# Autodesk Inventor assembly: SC40 700 Assembly
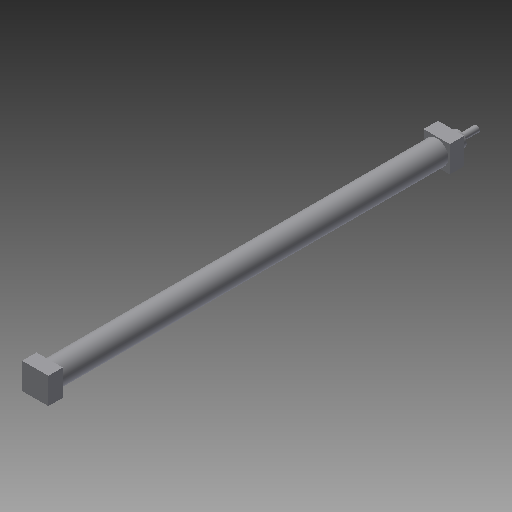
[picture p0: Inventor's stored thumbnail of the model, 512x512]
Saved by Autodesk Inventor 2019.4 (Build 234330000, 330)
## iProperties
Created: 2020-01-10
Part Number: SC40 700 Assembly
Document SubType Name: Assembly
Designer: Mark
Mass: 1404.85 g
Surface Area: 1514.62 cm^2
Volume: 1404.85 cm^3
Density: 1 g/cm^3
Author: Mark
## Documents named in this file (3)
- C:\Users\Mark\Desktop\7738 Helion Engineering\7738-2020\Elevator Mechanism\SC40 700 Assembly.iam
- C:\Users\Mark\Desktop\7738 Helion Engineering\7738-2020\Elevator Mechanism\SC40-700.ipt
- C:\Users\Mark\Desktop\7738 Helion Engineering\7738-2020\Elevator Mechanism\Bore.ipt
## Components (2 placed, 2 different names)
1. SC40-700:1 — Cylindrical:1
2. Bore:1 — Cylindrical:1
## Relationships (1: CylindricalJoint 1)
- Cylindrical:1: SC40-700:1 ↔ Bore:1
